# Autodesk Inventor assembly: om_Drop
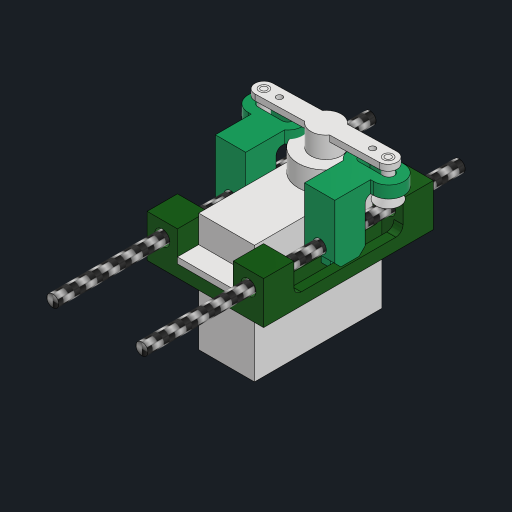
[picture p0: Inventor's stored thumbnail of the model, 512x512]
Saved by Autodesk Inventor 2023 (Build 270158000, 158)
## iProperties
Created: 2022-06-20
Part Number: om_Drop
Document SubType Name: Assembly
Designer: legot
Author: legot
## Documents named in this file (8)
- C:\Users\legot\Documents\Inventor\HIKOSAPO\Drop\om_Drop.iam
- C:\Users\legot\Documents\Inventor\HIKOSAPO\Drop\om_DropBase.ipt
- C:\Users\legot\Documents\Inventor\HIKOSAPO\Drop\om_Drop_R.ipt
- C:\Users\legot\Documents\Inventor\HIKOSAPO\Drop\om_Drop_L.ipt
- C:\Users\legot\Documents\Inventor\HIKOSAPO\public_parts\Horn.ipt
- C:\Users\legot\Documents\Inventor\HIKOSAPO\Drop\om_Drop_shaft.ipt
- C:\Users\legot\Documents\Inventor\HIKOSAPO\Drop\neji.ipt
- C:\Users\legot\Documents\Inventor\HIKOSAPO\public_parts\ServoMotor.ipt
## Components (9 placed, 7 different names)
1. om_DropBase:1 — メイト:7, メイト:9, フラッシュ:1, フラッシュ:2, メイト:12, メイト:13, メイト:14, 角度:1
2. om_Drop_R — メイト:9, メイト:10, 挿入:7, フラッシュ:2
3. om_Drop_L — メイト:7, メイト:11, 挿入:6, フラッシュ:1
4. Horn:1 — メイト:10, メイト:11, 挿入:4, 挿入:5, 挿入:8, 角度:1
5. om_Drop_shaft:1 — 挿入:7
6. om_Drop_shaft:2 — 挿入:6
7. neji:1 — 挿入:5
8. neji:2 — 挿入:4
9. ServoMotor:1 — メイト:12, メイト:13, メイト:14, 挿入:8
## Relationships (15: Mate 7, Insert 5, Flush 2, Angle 1)
- メイト:7 [Mate]: om_DropBase:1 ↔ om_Drop_L
- メイト:9 [Mate]: om_DropBase:1 ↔ om_Drop_R
- メイト:10 [Mate]: om_Drop_R ↔ Horn:1
- メイト:11 [Mate]: om_Drop_L ↔ Horn:1
- 挿入:4 [Insert]: Horn:1 ↔ neji:2
- 挿入:5 [Insert]: Horn:1 ↔ neji:1
- 挿入:6 [Insert] (18 mm): om_Drop_L ↔ om_Drop_shaft:2
- 挿入:7 [Insert] (-18 mm): om_Drop_R ↔ om_Drop_shaft:1
- フラッシュ:1 [Flush]: om_DropBase:1 ↔ om_Drop_L
- フラッシュ:2 [Flush]: om_DropBase:1 ↔ om_Drop_R
- メイト:12 [Mate]: om_DropBase:1 ↔ ServoMotor:1
- メイト:13 [Mate]: om_DropBase:1 ↔ ServoMotor:1
- メイト:14 [Mate]: om_DropBase:1 ↔ ServoMotor:1
- 挿入:8 [Insert]: Horn:1 ↔ ServoMotor:1
- 角度:1 [Angle] (0 deg): om_DropBase:1 ↔ Horn:1
